# Autodesk Inventor assembly: Assembly
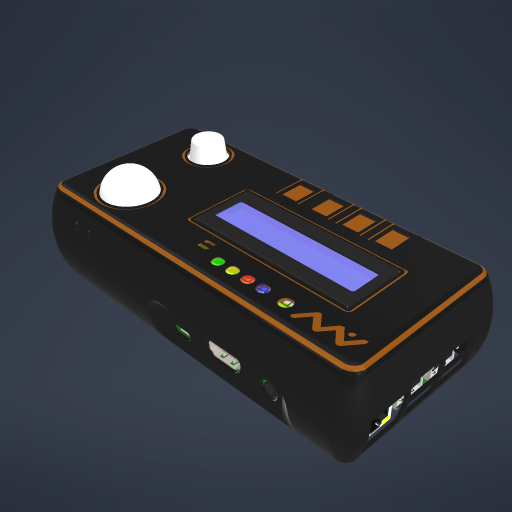
[picture p0: Inventor's stored thumbnail of the model, 512x512]
Saved by Autodesk Inventor 2023 (Build 270158000, 158)
## iProperties
Created: 2022-12-07
Part Number: Assembly
Document SubType Name: Assembly
Designer: Manuel
Author: Manuel
## Documents named in this file (8)
- C:\workspace\Studium\WST\opcua_netzwerk\Entwicklung Knoten\3D Modell\Assembly.iam
- C:\workspace\Studium\WST\opcua_netzwerk\Entwicklung Knoten\3D Modell\ConnectorHead_RPi\ConnectorHead_RPi.iam
- C:\workspace\Studium\WST\opcua_netzwerk\Entwicklung Knoten\3D Modell\Raspberry Pi 3B\Raspberry Pi 3.iam
- C:\workspace\Studium\WST\opcua_netzwerk\Entwicklung Knoten\3D Modell\16x2 LCD Display\LCD.iam
- C:\workspace\Studium\WST\opcua_netzwerk\Entwicklung Knoten\3D Modell\Case\Case.iam
- C:\workspace\Studium\WST\opcua_netzwerk\Entwicklung Knoten\3D Modell\Bewegungsmelder\pir-hc-sr-501-sensor.iam
- C:\workspace\Studium\WST\opcua_netzwerk\Entwicklung Knoten\3D Modell\BME280\Adafruit BME280.iam
- C:\workspace\Studium\WST\opcua_netzwerk\Entwicklung Knoten\3D Modell\MQ135\MQ135.iam
## Components (7 placed, 7 different names)
1. Raspberry Pi 3:1 [sub-assembly] — Passend:19, Passend:20, Passend:24
2. ConnectorHead_RPi:1 [sub-assembly] — Passend:15, Passend:16, Passend:22, Passend:23
3. LCD:1 [sub-assembly] — Passend:17, Passend:18, Passend:21
4. Case:1 [sub-assembly] — Passend:7, Passend:8, Passend:9, Passend:10, Passend:11, Winkel:1, Passend:12, Passend:13, Passend:14, Passend:15, Passend:16, Passend:17, Passend:18, Passend:19, Passend:20, Passend:21, Passend:22, Passend:23, Passend:24
5. pir-hc-sr-501-sensor:1 [sub-assembly] — Passend:7, Passend:8, Passend:9
6. Adafruit BME280:1 [sub-assembly] — Passend:12, Passend:13, Passend:14
7. MQ135:1 [sub-assembly] — Passend:10, Passend:11, Winkel:1
## Relationships (19: Mate 18, Angle 1)
- Passend:7 [Mate]: Case:1 ↔ pir-hc-sr-501-sensor:1
- Passend:8 [Mate]: Case:1 ↔ pir-hc-sr-501-sensor:1
- Passend:9 [Mate]: Case:1 ↔ pir-hc-sr-501-sensor:1
- Passend:10 [Mate]: Case:1 ↔ MQ135:1
- Passend:11 [Mate]: Case:1 ↔ MQ135:1
- Winkel:1 [Angle] (180 deg): Case:1 ↔ MQ135:1
- Passend:12 [Mate]: Case:1 ↔ Adafruit BME280:1
- Passend:13 [Mate]: Case:1 ↔ Adafruit BME280:1
- Passend:14 [Mate]: Case:1 ↔ Adafruit BME280:1
- Passend:15 [Mate]: ConnectorHead_RPi:1 ↔ Case:1
- Passend:16 [Mate]: ConnectorHead_RPi:1 ↔ Case:1
- Passend:17 [Mate]: LCD:1 ↔ Case:1
- Passend:18 [Mate]: LCD:1 ↔ Case:1
- Passend:19 [Mate]: Raspberry Pi 3:1 ↔ Case:1
- Passend:20 [Mate]: Raspberry Pi 3:1 ↔ Case:1
- Passend:21 [Mate]: LCD:1 ↔ Case:1
- Passend:22 [Mate]: ConnectorHead_RPi:1 ↔ Case:1
- Passend:23 [Mate]: ConnectorHead_RPi:1 ↔ Case:1
- Passend:24 [Mate]: Raspberry Pi 3:1 ↔ Case:1
